# Autodesk Inventor assembly: Flexipod2.0_2021_1_6
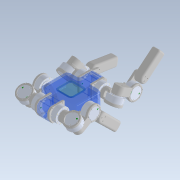
[picture p0: Inventor's stored thumbnail of the model, 180x180]
Saved by Autodesk Inventor 2020 (Build 240168000, 168)
## iProperties
Created: 2021-01-06
Part Number: Flexipod2.0_2021_1_6
Document SubType Name: Assembly
Designer: DELL
Author: DELL
## Documents named in this file (10)
- F:\SoftRobot2.0\FlexipodHardware2.0\FlexipodHardware\Flexipod2.0\robot_2021_1_6\Flexipod2.0_2021_1_6.iam
- F:\SoftRobot2.0\FlexipodHardware2.0\FlexipodHardware\Flexipod2.0\robot_2021_1_6\body.ipt
- F:\SoftRobot2.0\FlexipodHardware2.0\FlexipodHardware\Flexipod2.0\robot_2021_1_6\hip_link_4.ipt
- F:\SoftRobot2.0\FlexipodHardware2.0\FlexipodHardware\Flexipod2.0\robot_2021_1_6\hip_link_4_mirror.ipt
- F:\SoftRobot2.0\FlexipodHardware2.0\FlexipodHardware\Flexipod2.0\RMD_X6_stator.ipt
- F:\SoftRobot2.0\FlexipodHardware2.0\FlexipodHardware\Flexipod2.0\RMD_X6_rotor.ipt
- F:\SoftRobot2.0\FlexipodHardware2.0\FlexipodHardware\Flexipod2.0\robot_2021_1_6\thigh_link.ipt
- F:\SoftRobot2.0\FlexipodHardware2.0\FlexipodHardware\Flexipod2.0\robot_2021_1_6\shank_link.ipt
- F:\SoftRobot2.0\FlexipodHardware2.0\FlexipodHardware\Flexipod2.0\robot_2021_1_6\shank_thigh_connector.ipt
- F:\SoftRobot2.0\FlexipodHardware2.0\FlexipodHardware\Flexipod2.0\robot_2021_1_6\thigh_mirror.ipt
## Components (41 placed, 9 different names)
1. body:1 — Flush:1, Mate:1, Flush:2, Mate:2, Mate:3, Mate:4, Mate:5, Mate:6, Mate:7, Mate:8, Mate:9, Mate:10, Angle:1, Angle:2, Angle:3, Angle:4
2. hip_link_4:1 — Mate:2, Mate:16, Mate:23, Mate:36, Mate:37, Mate:38
3. hip_link_4:2 — Mate:18, Mate:19, Mate:20, Mate:27, Mate:28, Mate:29
4. hip_link_4_mirror:1 — Mate:15, Mate:24, Mate:25, Mate:39, Mate:40, Mate:41
5. hip_link_4_mirror:2 — Mate:17, Mate:21, Mate:22, Mate:33, Mate:34, Mate:35
6. RMD_X6_stator:1 — Mate:3, Mate:4, Mate:13, Flush:5
7. RMD_X6_stator:2 — Mate:7, Mate:8, Mate:12, Flush:4, Mate:22
8. RMD_X6_stator:3 — Mate:5, Mate:6, Mate:14, Flush:6, Mate:25
9. RMD_X6_stator:4 — Mate:9, Mate:10, Mate:11, Flush:3, Mate:20
10. RMD_X6_rotor:1 — Mate:12, Flush:4, Mate:17, Mate:21
11. RMD_X6_rotor:2 — Mate:13, Flush:5, Mate:16, Mate:23
12. RMD_X6_rotor:3 — Mate:14, Flush:6, Mate:15, Mate:24
13. RMD_X6_rotor:4 — Mate:11, Flush:3, Mate:18, Mate:19
14. RMD_X6_stator:5 — Mate:27, Mate:28, Mate:29, Angle:1, Mate:106
15. RMD_X6_rotor:5 — Mate:107, Mate:108
16. RMD_X6_stator:6 — Mate:33, Mate:34, Mate:35, Angle:2, Mate:100
17. RMD_X6_rotor:6 — Mate:101, Mate:102
18. RMD_X6_stator:7 — Mate:36, Mate:37, Mate:38, Angle:4, Mate:97
19. RMD_X6_rotor:7 — Mate:98, Mate:99
20. RMD_X6_stator:8 — Mate:39, Mate:40, Mate:41, Angle:3, Mate:114
21. RMD_X6_rotor:8 — Mate:115, Mate:116
22. RMD_X6_stator:9 — Mate:80, Mate:94, Mate:95, Mate:96
23. RMD_X6_rotor:9 — Mate:79, Mate:81
24. RMD_X6_stator:10 — Mate:77, Mate:111, Mate:112, Mate:113
25. RMD_X6_rotor:10 — Mate:76, Mate:78
26. RMD_X6_stator:11 — Mate:74, Mate:109, Mate:110
27. RMD_X6_rotor:11 — Mate:73, Mate:75
28. RMD_X6_stator:12 — Mate:72, Mate:103, Mate:104, Mate:105
29. RMD_X6_rotor:12 — Mate:70, Mate:71
30. shank_link:1 — Mate:88, Mate:89, Mate:90
31. shank_link:2 — Mate:82, Mate:83, Mate:84
32. shank_link:3 — Mate:85, Mate:86, Mate:87
33. shank_link:4 — Mate:91, Mate:92, Mate:93
34. shank_thigh_connector:1 — Mate:70, Mate:71, Mate:72, Mate:88, Mate:89, Mate:90
35. shank_thigh_connector:3 — Mate:73, Mate:74, Mate:75, Mate:91, Mate:92, Mate:93
36. shank_thigh_connector:4 — Mate:76, Mate:77, Mate:78, Mate:85, Mate:86, Mate:87
37. shank_thigh_connector:5 — Mate:79, Mate:80, Mate:81, Mate:82, Mate:83, Mate:84
38. thigh_link:1 — Mate:94, Mate:95, Mate:96, Mate:97, Mate:98, Mate:99
39. thigh_link:2 — Mate:106, Mate:107, Mate:108, Mate:109, Mate:110
40. thigh_mirror:1 — Mate:111, Mate:112, Mate:113, Mate:114, Mate:115, Mate:116
41. thigh_mirror:2 — Mate:100, Mate:101, Mate:102, Mate:103, Mate:104, Mate:105
## Relationships (110: Mate 92, Flush 14, Angle 4)
- Flush:1: body:1
- Mate:1: body:1
- Flush:2: body:1
- Mate:2: body:1 ↔ hip_link_4:1
- Mate:3: body:1 ↔ RMD_X6_stator:1
- Mate:4: body:1 ↔ RMD_X6_stator:1
- Mate:5: body:1 ↔ RMD_X6_stator:3
- Mate:6: body:1 ↔ RMD_X6_stator:3
- Mate:7: body:1 ↔ RMD_X6_stator:2
- Mate:8: body:1 ↔ RMD_X6_stator:2
- Mate:9: body:1 ↔ RMD_X6_stator:4
- Mate:10: body:1 ↔ RMD_X6_stator:4
- Mate:11: RMD_X6_stator:4 ↔ RMD_X6_rotor:4
- Flush:3 (-3 mm): RMD_X6_stator:4 ↔ RMD_X6_rotor:4
- Mate:12: RMD_X6_stator:2 ↔ RMD_X6_rotor:1
- Flush:4 (-3 mm): RMD_X6_stator:2 ↔ RMD_X6_rotor:1
- Mate:13: RMD_X6_stator:1 ↔ RMD_X6_rotor:2
- Flush:5 (-3 mm): RMD_X6_stator:1 ↔ RMD_X6_rotor:2
- Mate:14: RMD_X6_stator:3 ↔ RMD_X6_rotor:3
- Flush:6 (-3 mm): RMD_X6_stator:3 ↔ RMD_X6_rotor:3
- Mate:15: hip_link_4_mirror:1 ↔ RMD_X6_rotor:3
- Mate:16: hip_link_4:1 ↔ RMD_X6_rotor:2
- Mate:17: hip_link_4_mirror:2 ↔ RMD_X6_rotor:1
- Mate:18: hip_link_4:2 ↔ RMD_X6_rotor:4
- Mate:19: hip_link_4:2 ↔ RMD_X6_rotor:4
- Mate:20: hip_link_4:2 ↔ RMD_X6_stator:4
- Mate:21: hip_link_4_mirror:2 ↔ RMD_X6_rotor:1
- Mate:22: hip_link_4_mirror:2 ↔ RMD_X6_stator:2
- Mate:23: hip_link_4:1 ↔ RMD_X6_rotor:2
- Mate:24: hip_link_4_mirror:1 ↔ RMD_X6_rotor:3
- Mate:25: hip_link_4_mirror:1 ↔ RMD_X6_stator:3
- [Mate]: RMD_X6_stator:5 ↔ RMD_X6_rotor:5
- [Flush] (-3 mm): RMD_X6_stator:5 ↔ RMD_X6_rotor:5
- Mate:27: hip_link_4:2 ↔ RMD_X6_stator:5
- Mate:28: hip_link_4:2 ↔ RMD_X6_stator:5
- Mate:29: hip_link_4:2 ↔ RMD_X6_stator:5
- [Mate]: RMD_X6_stator:6 ↔ RMD_X6_rotor:6
- [Flush] (-3 mm): RMD_X6_stator:6 ↔ RMD_X6_rotor:6
- [Mate]: RMD_X6_stator:7 ↔ RMD_X6_rotor:7
- [Flush] (-3 mm): RMD_X6_stator:7 ↔ RMD_X6_rotor:7
- [Mate]: RMD_X6_stator:8 ↔ RMD_X6_rotor:8
- [Flush] (-3 mm): RMD_X6_stator:8 ↔ RMD_X6_rotor:8
- Mate:33: hip_link_4_mirror:2 ↔ RMD_X6_stator:6
- Mate:34: hip_link_4_mirror:2 ↔ RMD_X6_stator:6
- Mate:35: hip_link_4_mirror:2 ↔ RMD_X6_stator:6
- Mate:36: hip_link_4:1 ↔ RMD_X6_stator:7
- Mate:37: hip_link_4:1 ↔ RMD_X6_stator:7
- Mate:38: hip_link_4:1 ↔ RMD_X6_stator:7
- Mate:39: hip_link_4_mirror:1 ↔ RMD_X6_stator:8
- Mate:40: hip_link_4_mirror:1 ↔ RMD_X6_stator:8
- Mate:41: hip_link_4_mirror:1 ↔ RMD_X6_stator:8
- Angle:1 (30 deg): body:1 ↔ RMD_X6_stator:5
- Angle:2 (60 deg): body:1 ↔ RMD_X6_stator:6
- Angle:3 (240 deg): body:1 ↔ RMD_X6_stator:8
- Angle:4 (120 deg): body:1 ↔ RMD_X6_stator:7
- [Mate]: RMD_X6_stator:9 ↔ RMD_X6_rotor:9
- [Flush] (-3 mm): RMD_X6_stator:9 ↔ RMD_X6_rotor:9
- [Mate]: RMD_X6_stator:10 ↔ RMD_X6_rotor:10
- [Flush] (-3 mm): RMD_X6_stator:10 ↔ RMD_X6_rotor:10
- [Mate]: RMD_X6_stator:11 ↔ RMD_X6_rotor:11
- [Flush] (-3 mm): RMD_X6_stator:11 ↔ RMD_X6_rotor:11
- [Mate]: RMD_X6_stator:12 ↔ RMD_X6_rotor:12
- [Flush] (-3 mm): RMD_X6_stator:12 ↔ RMD_X6_rotor:12
- Mate:70: RMD_X6_rotor:12 ↔ shank_thigh_connector:1
- Mate:71: RMD_X6_rotor:12 ↔ shank_thigh_connector:1
- Mate:72: RMD_X6_stator:12 ↔ shank_thigh_connector:1
- Mate:73: RMD_X6_rotor:11 ↔ shank_thigh_connector:3
- Mate:74: RMD_X6_stator:11 ↔ shank_thigh_connector:3
- Mate:75: RMD_X6_rotor:11 ↔ shank_thigh_connector:3
- Mate:76: RMD_X6_rotor:10 ↔ shank_thigh_connector:4
- Mate:77: RMD_X6_stator:10 ↔ shank_thigh_connector:4
- Mate:78: RMD_X6_rotor:10 ↔ shank_thigh_connector:4
- Mate:79: RMD_X6_rotor:9 ↔ shank_thigh_connector:5
- Mate:80: RMD_X6_stator:9 ↔ shank_thigh_connector:5
- Mate:81: RMD_X6_rotor:9 ↔ shank_thigh_connector:5
- Mate:82: shank_link:2 ↔ shank_thigh_connector:5
- Mate:83: shank_link:2 ↔ shank_thigh_connector:5
- Mate:84: shank_link:2 ↔ shank_thigh_connector:5
- Mate:85: shank_link:3 ↔ shank_thigh_connector:4
- Mate:86: shank_link:3 ↔ shank_thigh_connector:4
- Mate:87: shank_link:3 ↔ shank_thigh_connector:4
- Mate:88: shank_link:1 ↔ shank_thigh_connector:1
- Mate:89: shank_link:1 ↔ shank_thigh_connector:1
- Mate:90: shank_link:1 ↔ shank_thigh_connector:1
- Mate:91: shank_link:4 ↔ shank_thigh_connector:3
- Mate:92: shank_link:4 ↔ shank_thigh_connector:3
- Mate:93: shank_link:4 ↔ shank_thigh_connector:3
- Mate:94: RMD_X6_stator:9 ↔ thigh_link:1
- Mate:95: RMD_X6_stator:9 ↔ thigh_link:1
- Mate:96: RMD_X6_stator:9 ↔ thigh_link:1
- Mate:97: RMD_X6_stator:7 ↔ thigh_link:1
- Mate:98: RMD_X6_rotor:7 ↔ thigh_link:1
- Mate:99: RMD_X6_rotor:7 ↔ thigh_link:1
- Mate:100: RMD_X6_stator:6 ↔ thigh_mirror:2
- Mate:101: RMD_X6_rotor:6 ↔ thigh_mirror:2
- Mate:102: RMD_X6_rotor:6 ↔ thigh_mirror:2
- Mate:103: RMD_X6_stator:12 ↔ thigh_mirror:2
- Mate:104: RMD_X6_stator:12 ↔ thigh_mirror:2
- Mate:105: RMD_X6_stator:12 ↔ thigh_mirror:2
- Mate:106: RMD_X6_stator:5 ↔ thigh_link:2
- Mate:107: RMD_X6_rotor:5 ↔ thigh_link:2
- Mate:108: RMD_X6_rotor:5 ↔ thigh_link:2
- Mate:109: RMD_X6_stator:11 ↔ thigh_link:2
- Mate:110: RMD_X6_stator:11 ↔ thigh_link:2
- Mate:111: RMD_X6_stator:10 ↔ thigh_mirror:1
- Mate:112: RMD_X6_stator:10 ↔ thigh_mirror:1
- Mate:113: RMD_X6_stator:10 ↔ thigh_mirror:1
- Mate:114: RMD_X6_stator:8 ↔ thigh_mirror:1
- Mate:115: RMD_X6_rotor:8 ↔ thigh_mirror:1
- Mate:116: RMD_X6_rotor:8 ↔ thigh_mirror:1
## Named parameters: d31_d14 = 0 mm, d32_d15 = -3 mm, d36_d31_d14 = 0 mm, d37_d32_d15 = -3 mm, d38_d31_d14 = 0 mm, d39_d32_d15 = -3 mm, d40_d31_d14 = 0 mm, d41_d32_d15 = -3 mm, d67_d36_d31_d14 = 0 mm, d68_d37_d32_d15 = -3 mm, d72_d67_d36_d31_d14 = 0 mm, d73_d68_d37_d32_d15 = -3 mm, d74_d67_d36_d31_d14 = 0 mm, d75_d68_d37_d32_d15 = -3 mm, d76_d67_d36_d31_d14 = 0 mm, d77_d68_d37_d32_d15 = -3 mm
